# Autodesk Inventor assembly: hipjoint_to_leg
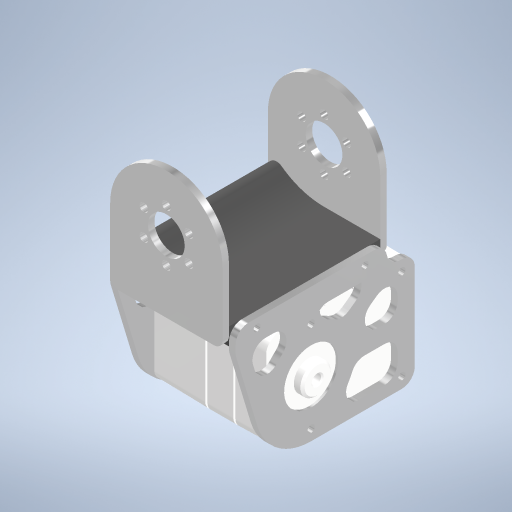
[picture p0: Inventor's stored thumbnail of the model, 512x512]
Saved by Autodesk Inventor 2024.1 (Build 281209000, 209)
## iProperties
Created: 2024-02-12
Part Number: hipjoint_to_leg
Document SubType Name: Assembly
Designer: hibik
Author: hibik
## Documents named in this file (5)
- C:\Users\hibik\Desktop\ロボメカ\HR\2024.02.11 Rl\02.11 ProtType\hipjoint_to_leg.iam
- C:\Users\hibik\Desktop\ロボメカ\HR\2024.02.11 Rl\02.11 ProtType\hipjoint_toleg_middle.ipt
- C:\Users\hibik\Desktop\ロボメカ\HR\2024.02.11 Rl\02.11 ProtType\hipjoint_toleg_upper.ipt
- C:\Users\hibik\Desktop\ロボメカ\HR\2024.02.11 Rl\KRS3300モータ.ipt
- C:\Users\hibik\Desktop\ロボメカ\HR\2024.02.11 Rl\02.11 ProtType\hipjoint_toleg_under.ipt
## Components (6 placed, 4 different names)
1. hipjoint_toleg_middle:1 — メイト:1, メイト:2, フラッシュ:1, フラッシュ:2, フラッシュ:3, フラッシュ:4, メイト:3, フラッシュ:5, フラッシュ:6
2. hipjoint_toleg_upper:1 — メイト:1, フラッシュ:3, フラッシュ:4
3. hipjoint_toleg_upper:2 — メイト:2, フラッシュ:1, フラッシュ:2
4. KRS3300モータ:1 — 挿入:1, 挿入:2, 角度:1, 角度:2
5. hipjoint_toleg_under:1 — 挿入:1, 角度:1, メイト:3, フラッシュ:5
6. hipjoint_toleg_under:2 — 挿入:2, 角度:2, フラッシュ:6
## Relationships (13: Flush 6, Mate 3, Insert 2, Angle 2)
- メイト:1 [Mate]: hipjoint_toleg_middle:1 ↔ hipjoint_toleg_upper:1
- メイト:2 [Mate]: hipjoint_toleg_middle:1 ↔ hipjoint_toleg_upper:2
- フラッシュ:1 [Flush]: hipjoint_toleg_middle:1 ↔ hipjoint_toleg_upper:2
- フラッシュ:2 [Flush]: hipjoint_toleg_middle:1 ↔ hipjoint_toleg_upper:2
- フラッシュ:3 [Flush]: hipjoint_toleg_middle:1 ↔ hipjoint_toleg_upper:1
- フラッシュ:4 [Flush]: hipjoint_toleg_middle:1 ↔ hipjoint_toleg_upper:1
- 挿入:1 [Insert]: KRS3300モータ:1 ↔ hipjoint_toleg_under:1
- 挿入:2 [Insert]: KRS3300モータ:1 ↔ hipjoint_toleg_under:2
- 角度:1 [Angle] (0 deg): KRS3300モータ:1 ↔ hipjoint_toleg_under:1
- 角度:2 [Angle] (0 deg): KRS3300モータ:1 ↔ hipjoint_toleg_under:2
- メイト:3 [Mate]: hipjoint_toleg_middle:1 ↔ hipjoint_toleg_under:1
- フラッシュ:5 [Flush]: hipjoint_toleg_middle:1 ↔ hipjoint_toleg_under:1
- フラッシュ:6 [Flush]: hipjoint_toleg_middle:1 ↔ hipjoint_toleg_under:2
